# Autodesk Inventor assembly: Assembly1
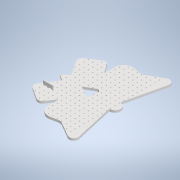
[picture p0: Inventor's stored thumbnail of the model, 180x180]
Saved by Autodesk Inventor 2020.2 (Build 242310000, 310)
## iProperties
Created: 2020-03-02
Part Number: Assembly1
Document SubType Name: Assembly
Designer: lenovo
Author: lenovo
## Documents named in this file (3)
- F:\siri\siri final\Assembly1.iam
- F:\siri\Butterfly(my own.3).ipt
- F:\siri\Bocks.ipt
## Components (3 placed, 2 different names)
1. Butterfly(my own.3):1 — Rotational:1, Rotational:2
2. Bocks:1 — Rotational:1
3. Bocks:2 — Rotational:2
## Relationships (2: RevoluteJoint 2)
- Rotational:1 [RevoluteJoint]: Butterfly(my own.3):1 ↔ Bocks:1
- Rotational:2 [RevoluteJoint]: Butterfly(my own.3):1 ↔ Bocks:2
